# Autodesk Inventor assembly: ALOHA2_viperx_v2
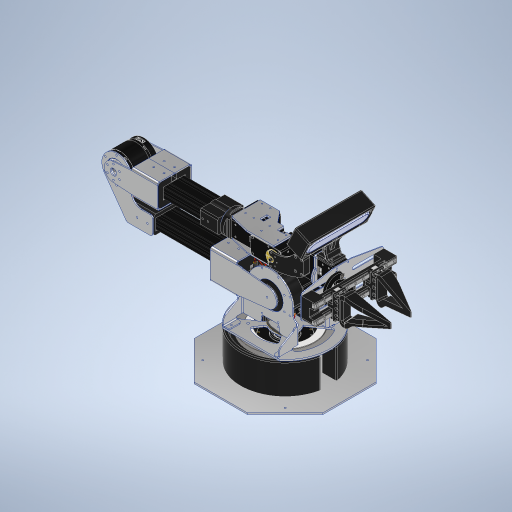
[picture p0: Inventor's stored thumbnail of the model, 512x512]
Saved by Autodesk Inventor 2024.3 (Build 283343010, 343A)
## iProperties
Created: 2025-10-05
Part Number: ALOHA2_viperx_v2
Document SubType Name: Assembly
Designer: kshau
Author: kshau
## Documents named in this file (6)
- C:\Users\kshau\Documents\inventor\Create_ViperX\Create_ViperX_ALOHA\ILOHA2_Arm.iam
- C:\Users\kshau\Documents\inventor\Create_ViperX\Create_ViperX_ALOHA\Base_Component_v2\Base_Component_v2.iam
- ArmBase_v2.iam
- C:\Users\kshau\Documents\inventor\Create_ViperX\Create_ViperX_ALOHA\UpperArm_Component_v2\UpperArm_v2.iam
- C:\Users\kshau\Documents\inventor\Create_ViperX\Create_ViperX_ALOHA\ForeArm_Component\ForeArm.iam
- C:\Users\kshau\Documents\inventor\Create_ViperX\Create_ViperX_ALOHA\VipperX_hommage_v2\AIP\ケーブル＆ハーネス\ILOHA2_Arm_v2.Harness1.iam
## Components (4 placed, 4 different names)
1. ArmBase_v2:1 [sub-assembly] — 回転:1, 回転:2, メイト:1, メイト:2, メイト:6
2. UpperArm_v2:1 [sub-assembly] — 回転:1, 回転:2, 回転:3, 回転:4, メイト:1, メイト:2, メイト:3, メイト:4, メイト:5, メイト:6
3. ForeArm:1 [sub-assembly] — 回転:3, 回転:4, メイト:3, メイト:4, メイト:5
4. Harness1 [sub-assembly]
## Relationships (10: Mate 6, RevoluteJoint 4)
- 回転:1 [RevoluteJoint]: ArmBase_v2:1 ↔ UpperArm_v2:1
- 回転:2 [RevoluteJoint]: ArmBase_v2:1 ↔ UpperArm_v2:1
- 回転:3 [RevoluteJoint]: UpperArm_v2:1 ↔ ForeArm:1
- 回転:4 [RevoluteJoint]: UpperArm_v2:1 ↔ ForeArm:1
- メイト:1 [Mate]: ArmBase_v2:1 ↔ UpperArm_v2:1
- メイト:2 [Mate]: ArmBase_v2:1 ↔ UpperArm_v2:1
- メイト:3 [Mate]: UpperArm_v2:1 ↔ ForeArm:1
- メイト:4 [Mate]: UpperArm_v2:1 ↔ ForeArm:1
- メイト:5 [Mate] (39.55 mm): UpperArm_v2:1 ↔ ForeArm:1
- メイト:6 [Mate] (5 mm): ArmBase_v2:1 ↔ UpperArm_v2:1
